# Autodesk Inventor assembly: aircilinder_100
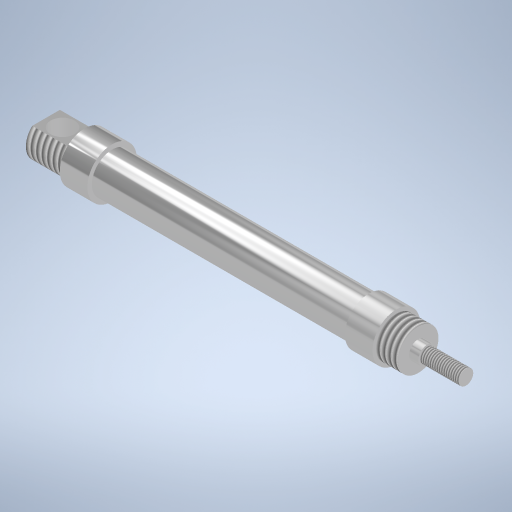
[picture p0: Inventor's stored thumbnail of the model, 512x512]
Saved by Autodesk Inventor 2024.1 (Build 281209000, 209)
## iProperties
Created: 2023-11-21
Part Number: aircilinder_100
Document SubType Name: Assembly
Designer: haruy
Author: haruy
## Documents named in this file (3)
- C:\Users\haruy\OneDrive - Kyushu University\KURT_工房共有\2023~2024\ハード\CAD\2024NHK\000_parts\エアシリンダー\airclinder\aircilinder_100.iam
- C:\Users\haruy\OneDrive - Kyushu University\KURT_工房共有\2023~2024\ハード\CAD\2024NHK\000_parts\エアシリンダー\airclinder\aircilinder_100_top.ipt
- C:\Users\haruy\OneDrive - Kyushu University\KURT_工房共有\2023~2024\ハード\CAD\2024NHK\000_parts\エアシリンダー\airclinder\aircilinder_100_under.ipt
## Components (2 placed, 2 different names)
1. aircilinder_100_top:1 — 円柱状:1
2. aircilinder_100_under:1 — 円柱状:1
## Relationships (1: CylindricalJoint 1)
- 円柱状:1 [CylindricalJoint]: aircilinder_100_top:1 ↔ aircilinder_100_under:1
